# Autodesk Inventor assembly: Servo-Arm-20mm-Enhanced-Ball-Joint
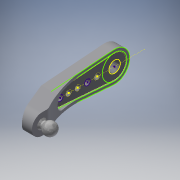
[picture p0: Inventor's stored thumbnail of the model, 180x180]
Saved by Autodesk Inventor 2018.2 (Build 222227000, 227)
## iProperties
Created: 2018-02-23
Part Number: Servo-Arm-20mm-Enhanced-Ball-Joint
Material: Generisch
Document SubType Name: Assembly
Designer: JochenAlt
Author: JochenAlt
## Documents named in this file (3)
- D:\Projects\Donna\CAD\KST DS215MG\Servo-Arm-20mm-Enhanced-Ball-Joint.iam
- D:\Projects\Donna\CAD\KST DS215MG\Ball-Joint-male.ipt
- D:\Projects\Donna\CAD\KST DS215MG\Servo-Arm-20mm-Enhanced.ipt
## Components (2 placed, 2 different names)
1. ball joint:1 — Passend:4, Passend:5
2. ServoArm:1 — Passend:1, Passend:2, Passend:3, Passend:4, Passend:5
## Relationships (5: Mate 5)
- Passend:1 [Mate]: ServoArm:1
- Passend:2 [Mate]: ServoArm:1
- Passend:3 [Mate]: ServoArm:1
- Passend:4 [Mate]: ball joint:1 ↔ ServoArm:1
- Passend:5 [Mate]: ball joint:1 ↔ ServoArm:1
